# Autodesk Inventor assembly: joint4
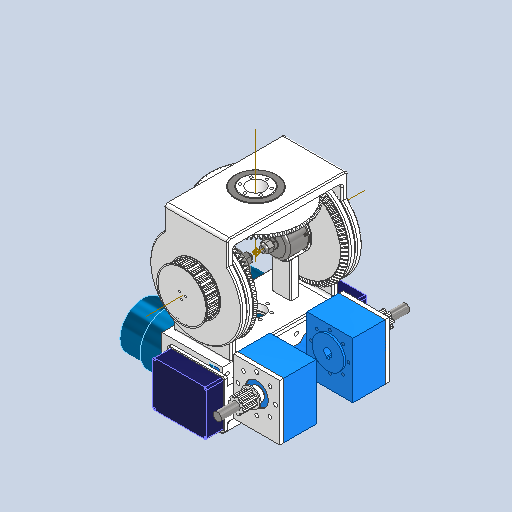
[picture p0: Inventor's stored thumbnail of the model, 512x512]
Saved by Autodesk Inventor 2025.3 (Build 293356030, 356C)
## iProperties
Created: 2025-08-31
Part Number: joint4
Document SubType Name: Assembly
Designer: MSI
Mass: 17501.7 g
Surface Area: 10758.8 cm^2
Volume: 6522.31 cm^3
Density: 2.68337 g/cm^3
Author: MSI
## Documents named in this file (14)
- C:\Users\MSI\Desktop\Project\3. 로봇팔\Robot Arm Model\Robot_Arm_6_v1\joint4.iam
- C:\Users\MSI\Desktop\Project\3. 로봇팔\Robot Arm Model\Robot_Arm_6_v1\miter_gear_center.ipt
- C:\Users\MSI\Desktop\Project\3. 로봇팔\Robot Arm Model\Robot_Arm_6_v1\miter_gear_left.ipt
- C:\Users\MSI\Desktop\Project\3. 로봇팔\Robot Arm Model\Robot_Arm_6_v1\miter_gear_right.ipt
- C:\Users\MSI\Desktop\Project\3. 로봇팔\Robot Arm Model\Robot_Arm_6_v1\encoder.ipt
- C:\Users\MSI\Desktop\Project\3. 로봇팔\Robot Arm Model\Robot_Arm_6_v1\belt_pulley_1.ipt
- C:\Users\MSI\Desktop\Project\3. 로봇팔\Robot Arm Model\Robot_Arm_6_v1\belt_pulley_2.ipt
- C:\Users\MSI\Desktop\Project\3. 로봇팔\Robot Arm Model\Robot_Arm_6_v1\encoder_frame.ipt
- C:\Users\MSI\Desktop\Project\3. 로봇팔\Robot Arm Model\Robot_Arm_6_v1\joint4_frame.ipt
- C:\Users\MSI\Desktop\Project\3. 로봇팔\Robot Arm Model\Robot_Arm_6_v1\motor.iam
- C:\Users\MSI\Desktop\Project\3. 로봇팔\Robot Arm Model\Robot_Arm_6_v1\C-E6704ZZ_Autodesk_Inventor_2024_20250921\C-E6704ZZ.ipt
- C:\Users\MSI\Desktop\Project\3. 로봇팔\Robot Arm Model\Robot_Arm_6_v1\joint4_base.ipt
- C:\Users\MSI\Desktop\Project\3. 로봇팔\Robot Arm Model\Robot_Arm_6_v1\C-E6810ZZ_Autodesk_Inventor_2024_20250921\C-E6810ZZ.ipt
- C:\Users\MSI\Desktop\Project\3. 로봇팔\Robot Arm Model\Robot_Arm_6_v1\NTN_GS81110OuterRings\GS81110Outer Rings.ipt
## Components (21 placed, 12 different names)
1. motor:1 [sub-assembly] — 강체:20, 강체:21, 강체:22
2. joint4_base:1 — 회전:1, 강체:15, 강체:17, 강체:22, 강체:25, 강체:26, 강체:18, 강체:19
3. joint4_frame:1 — 회전:1, 회전:4, 강체:23, 강체:24, 강체:27, 강체:28, 강체:29
4. 베벨 기어2:1 — 회전:4
5. 베벨 기어1:1 — 강체:18, 강체:8
6. 베벨 기어1:2 — 강체:19, 강체:6
7. encoder:1 — 강체:16
8. encoder:2 — 강체:14
9. 동기식 풀리1:1 — 강체:20
10. 동기식 풀리2:1 — 강체:6
11. 동기식 풀리1:2 — 강체:21
12. 동기식 풀리2:2 — 강체:8
13. encoder_frame:1 — 강체:14, 강체:15
14. encoder_frame:2 — 강체:16, 강체:17
15. C-E6704ZZ:1 — 강체:23
16. C-E6704ZZ:2 — 강체:24
17. C-E6704ZZ:3 — 강체:26
18. C-E6704ZZ:4 — 강체:25
19. C-E6810ZZ:1 — 강체:27
20. GS81110Outer Rings:1 — 강체:29
21. GS81110Outer Rings:2 — 강체:28
## Relationships (20: WeldJoint 18, RevoluteJoint 2)
- 회전:1 [RevoluteJoint] (-1 mm): joint4_base:1 ↔ joint4_frame:1
- 강체:18 [WeldJoint] (-1 mm): joint4_base:1 ↔ 베벨 기어1:1
- 강체:19 [WeldJoint] (-1 mm): joint4_base:1 ↔ 베벨 기어1:2
- 회전:4 [RevoluteJoint] (-1 mm): joint4_frame:1 ↔ 베벨 기어2:1
- 강체:16 [WeldJoint]: encoder:1 ↔ encoder_frame:2
- 강체:14 [WeldJoint]: encoder:2 ↔ encoder_frame:1
- 강체:6 [WeldJoint]: 베벨 기어1:2 ↔ 동기식 풀리2:1
- 강체:8 [WeldJoint]: 베벨 기어1:1 ↔ 동기식 풀리2:2
- 강체:15 [WeldJoint]: joint4_base:1 ↔ encoder_frame:1
- 강체:17 [WeldJoint]: joint4_base:1 ↔ encoder_frame:2
- 강체:20 [WeldJoint]: motor:1 ↔ 동기식 풀리1:1
- 강체:21 [WeldJoint]: motor:1 ↔ 동기식 풀리1:2
- 강체:22 [WeldJoint]: motor:1 ↔ joint4_base:1
- 강체:23 [WeldJoint]: joint4_frame:1 ↔ C-E6704ZZ:1
- 강체:24 [WeldJoint]: joint4_frame:1 ↔ C-E6704ZZ:2
- 강체:25 [WeldJoint]: joint4_base:1 ↔ C-E6704ZZ:4
- 강체:26 [WeldJoint]: joint4_base:1 ↔ C-E6704ZZ:3
- 강체:27 [WeldJoint] (-1 mm): joint4_frame:1 ↔ C-E6810ZZ:1
- 강체:28 [WeldJoint]: joint4_frame:1 ↔ GS81110Outer Rings:2
- 강체:29 [WeldJoint]: joint4_frame:1 ↔ GS81110Outer Rings:1
